# Autodesk Inventor assembly: 2.75 Omni AS, No Insert_mirrored
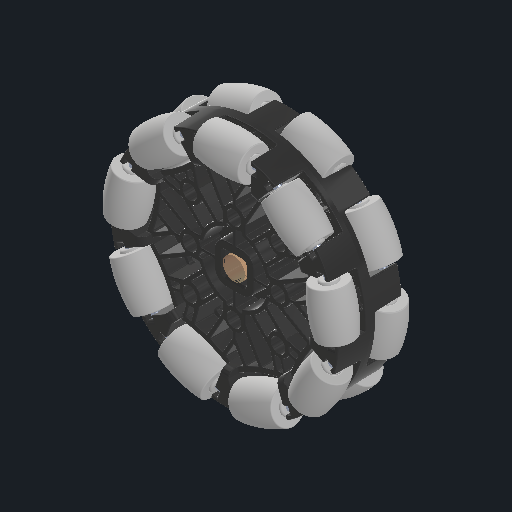
[picture p0: Inventor's stored thumbnail of the model, 512x512]
Saved by Autodesk Inventor 2025 (Build 290162000, 162)
## iProperties
Created: 2022-08-02
Part Number: 2.75 Omni AS, No Insert_mirrored
Document SubType Name: Assembly
Designer: Averey Ku
Author: ylu12
## Documents named in this file (2)
- D:\vex_robotics_high_stakes\hardware\cad\EARLY_SEASON\chassis\mirrored_parts\2.75 Omni AS, No Insert_mirrored.iam
- D:\vex_robotics_high_stakes\hardware\cad\EARLY_SEASON\chassis\mirrored_parts\2.75 Omni Antistatic_mirrored.ipt
## Components (1 placed, 1 different names)
1. 2.75 Omni Antistatic_mirrored:1 — Mate:8, Mate:7, Flush:4
## Relationships (3: Mate 2, Flush 1)
- Mate:8: 2.75 Omni Antistatic_mirrored:1
- Mate:7: 2.75 Omni Antistatic_mirrored:1
- Flush:4: 2.75 Omni Antistatic_mirrored:1
